# Autodesk Inventor assembly: Pass_Fail_Rig_v2
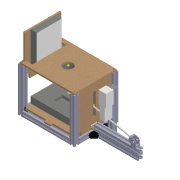
[picture p0: Inventor's stored thumbnail of the model, 180x180]
Saved by Autodesk Inventor 2021 (Build 250183000, 183)
## iProperties
Created: 2021-02-17
Part Number: Pass_Fail_Rig_v2
Document SubType Name: Assembly
Designer: negt20
Author: negt20
## Documents named in this file (23)
- C:\Users\negt20\OneDrive - University of Bath\Documents\Inventor\Pass_Fail_Rig\New Rig\Pass_Fail_Rig_v2.iam
- C:\Users\negt20\OneDrive - University of Bath\Documents\Inventor\Pass_Fail_Rig\New Rig\Strut_Profile_20x20_width.ipt
- C:\Users\negt20\OneDrive - University of Bath\Documents\Inventor\Pass_Fail_Rig\New Rig\Strut_Profile_20x20_height.ipt
- C:\Users\negt20\OneDrive - University of Bath\Documents\Inventor\Pass_Fail_Rig\New Rig\Strut_Profile_20x20_length.ipt
- C:\Users\negt20\OneDrive - University of Bath\Documents\Inventor\Pass_Fail_Rig\New Rig\Inner_Bracket_6mm.ipt
- C:\Users\negt20\OneDrive - University of Bath\Documents\Inventor\Pass_Fail_Rig\New Rig\Outer_Bracket_20x20.ipt
- C:\Users\negt20\OneDrive - University of Bath\Documents\Inventor\Pass_Fail_Rig\New Rig\Strut_Profile_20x20_pivotlength.ipt
- C:\Users\negt20\OneDrive - University of Bath\Documents\Inventor\Pass_Fail_Rig\New Rig\MDF_Hammer_Side.ipt
- C:\Users\negt20\OneDrive - University of Bath\Documents\Inventor\Pass_Fail_Rig\New Rig\Threaded hammer.ipt
- C:\Users\negt20\OneDrive - University of Bath\Documents\Inventor\Pass_Fail_Rig\New Rig\MDF_Side.ipt
- C:\Users\negt20\OneDrive - University of Bath\Documents\Inventor\Pass_Fail_Rig\New Rig\MDF_Front.ipt
- C:\Users\negt20\OneDrive - University of Bath\Documents\Inventor\Pass_Fail_Rig\New Rig\MDF_Base.ipt
- C:\Users\negt20\OneDrive - University of Bath\Documents\Inventor\Pass_Fail_Rig\New Rig\Foam_Side.ipt
- C:\Users\negt20\OneDrive - University of Bath\Documents\Inventor\Pass_Fail_Rig\New Rig\Foam_Hammer_Side.ipt
- C:\Users\negt20\OneDrive - University of Bath\Documents\Inventor\Pass_Fail_Rig\New Rig\Foam_Front.ipt
- C:\Users\negt20\OneDrive - University of Bath\Documents\Inventor\Pass_Fail_Rig\New Rig\Foam_Base.ipt
- C:\Users\negt20\OneDrive - University of Bath\Documents\Inventor\Pass_Fail_Rig\New Rig\MDF_Top_Big_Mic.ipt
- C:\Users\negt20\OneDrive - University of Bath\Documents\Inventor\Pass_Fail_Rig\New Rig\Foam_Top_Big_Mic.ipt
- C:\Users\negt20\OneDrive - University of Bath\Documents\Inventor\Pass_Fail_Rig\New Rig\MDF_Top_Small_Mics.ipt
- C:\Users\negt20\OneDrive - University of Bath\Documents\Inventor\Pass_Fail_Rig\New Rig\Foam_Top_Small_Mics.ipt
- C:\Users\negt20\OneDrive - University of Bath\Documents\Inventor\Pass_Fail_Rig\New Rig\T_NUT_N6.ipt
- C:\Users\negt20\OneDrive - University of Bath\Documents\Inventor\Pass_Fail_Rig\New Rig\Actuator.ipt
- C:\Users\negt20\OneDrive - University of Bath\Documents\Inventor\Pass_Fail_Rig\New Rig\JOINT_20X20_detail.iam
## Components (57 placed, 22 different names)
1. Outer_Bracket_20x20:9 — Mate:104, Mate:105
2. Outer_Bracket_20x20:10 — Mate:106, Mate:107
3. Outer_Bracket_20x20:11 — Mate:108, Mate:109
4. Outer_Bracket_20x20:12 — Mate:110, Mate:111
5. Strut_Profile_20x20_height:1 — Mate:1, Flush:1, Flush:2, Flush:7, Mate:13, Mate:15, Mate:36, Flush:17, Mate:49, Mate:52, Mate:53, Mate:55, Mate:57, Mate:71, Insert:4, Insert:8, Mate:88
6. Strut_Profile_20x20_width:1 — Mate:1, Flush:1, Flush:2, Mate:2, Flush:3, Flush:4, Mate:3, Flush:6, Flush:8, Mate:21, Mate:22, Mate:30, Mate:31, Mate:45, Mate:46, Mate:54, Mate:4, Mate:98, Flush:24, Mate:104, Mate:110
7. Strut_Profile_20x20_height:2 — Mate:2, Flush:3, Flush:4, Flush:5, Mate:18, Mate:26, Mate:35, Flush:15, Flush:16, Mate:47, Mate:51, Mate:59, Mate:62, Mate:67, Mate:68, Mate:74, Mate:79, Insert:2, Insert:7, Mate:97
8. Strut_Profile_20x20_length:1 — Mate:3, Flush:5, Flush:6, Mate:6, Flush:11, Flush:12, Mate:23, Mate:24, Mate:32, Mate:34, Mate:61
9. Strut_Profile_20x20_length:2 — Mate:4, Flush:7, Flush:8, Mate:5, Flush:9, Flush:10, Mate:19, Mate:20, Mate:27, Mate:29, Flush:18, Mate:58, Mate:66
10. Strut_Profile_20x20_height:3 — Mate:5, Flush:9, Flush:10, Mate:7, Mate:11, Mate:12, Mate:56, Mate:63, Mate:64, Insert:3, Insert:5, Mate:96
11. Strut_Profile_20x20_height:4 — Mate:6, Flush:11, Flush:12, Mate:8, Flush:13, Flush:14, Mate:16, Mate:17, Mate:60, Mate:78, Insert:1, Insert:6, Mate:95
12. Strut_Profile_20x20_width:2 — Mate:7, Mate:8, Flush:13, Flush:14, Mate:10, Mate:25, Mate:28, Mate:33, Mate:65-door
13. T_NUT_N6:1 — Insert:9
14. T_NUT_N6:2 — Insert:12
15. T_NUT_N6:3 — Insert:10
16. T_NUT_N6:4 — Insert:11
17. Inner_Bracket_6mm:1 — Mate:10, Mate:11, Mate:96
18. Inner_Bracket_6mm:2 — Mate:13, Mate:22
19. Inner_Bracket_6mm:3 — Mate:12, Mate:20
20. Inner_Bracket_6mm:4 — Mate:16, Mate:24, Mate:78
21. Inner_Bracket_6mm:5 — Mate:17, Mate:25, Mate:95
22. Inner_Bracket_6mm:6 — Mate:18, Mate:21
23. Inner_Bracket_6mm:7 — Mate:15, Mate:19
24. Inner_Bracket_6mm:8 — Mate:23, Mate:26, Mate:79
25. Outer_Bracket_20x20:1 — Mate:27, Mate:28
26. Outer_Bracket_20x20:2 — Mate:29, Mate:30
27. Outer_Bracket_20x20:3 — Mate:31, Mate:32
28. Outer_Bracket_20x20:4 — Mate:33, Mate:34
29. MDF_Top_Big_Mic:1 — Insert:1, Insert:2, Insert:3, Insert:4, Mate:86
30. MDF_Top_Small_Mics:1 — Insert:5, Insert:6, Insert:7, Insert:8, Mate:88
31. MDF_Base:1 — Mate:66, Mate:67, Mate:68, Mate:70, Mate:73, Mate:76, Mate:83, Insert:9, Insert:10, Insert:11, Insert:12
32. MDF_Side:1 — Mate:55, Mate:56, Mate:57, Mate:58, Mate:69
33. MDF_Hammer_Side:1 — Mate:51, Mate:52, Mate:53, Mate:54, Mate:75, Flush:27
34. MDF_Front:1 — Mate:63, Mate:64, Mate:65-door, Mate:80, Flush:22
35. MDF_Side:2 — Mate:59, Mate:60, Mate:61, Mate:62, Mate:72
36. Foam_Top_Big_Mic:1 — Mate:86, Mate:87, Mate:91
37. Foam_Top_Small_Mics:1 — Mate:89, Mate:90, Flush:23
38. Foam_Base:1 — Mate:83, Mate:84, Mate:93
39. Foam_Side:1 — Mate:69, Mate:70, Mate:71, Mate:90, Mate:91, Mate:92, Mate:93, Mate:94
40. Foam_Hammer_Side:1 — Mate:75, Mate:76, Mate:84, Mate:87, Mate:89, Flush:23, Mate:94
41. Foam_Front:1 — Mate:80, Flush:22, Mate:92
42. Foam_Side:2 — Mate:72, Mate:73, Mate:74
43. Strut_Profile_20x20_pivotlength:1 — Mate:35, Flush:15, Flush:16, Mate:37, Flush:19, Flush:20, Mate:39, Mate:41, Mate:48
44. Strut_Profile_20x20_pivotlength:2 — Mate:36, Flush:17, Flush:18, Mate:38, Mate:40, Mate:42, Mate:50
45. Strut_Profile_20x20_width:3 — Mate:37, Mate:38, Flush:19, Flush:20, Mate:43, Mate:44
46. Outer_Bracket_20x20:5 — Mate:40, Mate:45
47. Outer_Bracket_20x20:6 — Mate:39, Mate:46
48. Outer_Bracket_20x20:7 — Mate:41, Mate:43
49. Outer_Bracket_20x20:8 — Mate:42, Mate:44
50. Inner_Bracket_6mm:9 — Mate:49, Mate:50
51. Inner_Bracket_6mm:10 — Mate:47, Mate:48, Mate:97
52. Threaded hammer:1 — Insert:13, Mate:103
53. Strut_Profile_20x20_pivotlength:3 — Mate:98, Flush:24, Mate:99, Flush:25, Flush:27, Flush:28, Flush:29, Mate:101, Mate:105, Mate:107, Mate:111
54. Strut_Profile_20x20_height:5 — Mate:99, Flush:25, Mate:100, Flush:26, Mate:106, Mate:109
55. Actuator:1 — Mate:100, Flush:26
56. Strut_Profile_20x20_pivotlength:4 — Flush:28, Flush:29, Mate:101, Mate:102, Mate:108
57. JOINT_20X20_detail:1 [sub-assembly] — Mate:102, Insert:13, Mate:103
## Relationships (146: Mate 105, Flush 28, Insert 13)
- Mate:1: Strut_Profile_20x20_height:1 ↔ Strut_Profile_20x20_width:1
- Flush:1: Strut_Profile_20x20_height:1 ↔ Strut_Profile_20x20_width:1
- Flush:2: Strut_Profile_20x20_height:1 ↔ Strut_Profile_20x20_width:1
- Mate:2: Strut_Profile_20x20_width:1 ↔ Strut_Profile_20x20_height:2
- Flush:3: Strut_Profile_20x20_width:1 ↔ Strut_Profile_20x20_height:2
- Flush:4: Strut_Profile_20x20_width:1 ↔ Strut_Profile_20x20_height:2
- Mate:3: Strut_Profile_20x20_width:1 ↔ Strut_Profile_20x20_length:1
- Flush:5: Strut_Profile_20x20_height:2 ↔ Strut_Profile_20x20_length:1
- Flush:6: Strut_Profile_20x20_width:1 ↔ Strut_Profile_20x20_length:1
- Mate:4: Strut_Profile_20x20_width:1 ↔ Strut_Profile_20x20_length:2
- Flush:7: Strut_Profile_20x20_height:1 ↔ Strut_Profile_20x20_length:2
- Flush:8: Strut_Profile_20x20_width:1 ↔ Strut_Profile_20x20_length:2
- Mate:5: Strut_Profile_20x20_length:2 ↔ Strut_Profile_20x20_height:3
- Flush:9: Strut_Profile_20x20_length:2 ↔ Strut_Profile_20x20_height:3
- Flush:10: Strut_Profile_20x20_length:2 ↔ Strut_Profile_20x20_height:3
- Mate:6: Strut_Profile_20x20_length:1 ↔ Strut_Profile_20x20_height:4
- Flush:11: Strut_Profile_20x20_length:1 ↔ Strut_Profile_20x20_height:4
- Flush:12: Strut_Profile_20x20_length:1 ↔ Strut_Profile_20x20_height:4
- Mate:7: Strut_Profile_20x20_height:3 ↔ Strut_Profile_20x20_width:2
- Mate:8: Strut_Profile_20x20_height:4 ↔ Strut_Profile_20x20_width:2
- Flush:13: Strut_Profile_20x20_height:4 ↔ Strut_Profile_20x20_width:2
- Flush:14: Strut_Profile_20x20_height:4 ↔ Strut_Profile_20x20_width:2
- Mate:10: Strut_Profile_20x20_width:2 ↔ Inner_Bracket_6mm:1
- Mate:11: Strut_Profile_20x20_height:3 ↔ Inner_Bracket_6mm:1
- Mate:12: Strut_Profile_20x20_height:3 ↔ Inner_Bracket_6mm:3
- Mate:13: Strut_Profile_20x20_height:1 ↔ Inner_Bracket_6mm:2
- Mate:15: Strut_Profile_20x20_height:1 ↔ Inner_Bracket_6mm:7
- Mate:16: Strut_Profile_20x20_height:4 ↔ Inner_Bracket_6mm:4
- Mate:17: Strut_Profile_20x20_height:4 ↔ Inner_Bracket_6mm:5
- Mate:18: Strut_Profile_20x20_height:2 ↔ Inner_Bracket_6mm:6
- Mate:19: Strut_Profile_20x20_length:2 ↔ Inner_Bracket_6mm:7
- Mate:20: Strut_Profile_20x20_length:2 ↔ Inner_Bracket_6mm:3
- Mate:21: Strut_Profile_20x20_width:1 ↔ Inner_Bracket_6mm:6
- Mate:22: Strut_Profile_20x20_width:1 ↔ Inner_Bracket_6mm:2
- Mate:23: Strut_Profile_20x20_length:1 ↔ Inner_Bracket_6mm:8
- Mate:24: Strut_Profile_20x20_length:1 ↔ Inner_Bracket_6mm:4
- Mate:25: Strut_Profile_20x20_width:2 ↔ Inner_Bracket_6mm:5
- Mate:26: Strut_Profile_20x20_height:2 ↔ Inner_Bracket_6mm:8
- Mate:27: Strut_Profile_20x20_length:2 ↔ Outer_Bracket_20x20:1
- Mate:28: Strut_Profile_20x20_width:2 ↔ Outer_Bracket_20x20:1
- Mate:29: Strut_Profile_20x20_length:2 ↔ Outer_Bracket_20x20:2
- Mate:30: Strut_Profile_20x20_width:1 ↔ Outer_Bracket_20x20:2
- Mate:31: Strut_Profile_20x20_width:1 ↔ Outer_Bracket_20x20:3
- Mate:32: Strut_Profile_20x20_length:1 ↔ Outer_Bracket_20x20:3
- Mate:33: Strut_Profile_20x20_width:2 ↔ Outer_Bracket_20x20:4
- Mate:34: Strut_Profile_20x20_length:1 ↔ Outer_Bracket_20x20:4
- Mate:35: Strut_Profile_20x20_height:2 ↔ Strut_Profile_20x20_pivotlength:1
- Flush:15: Strut_Profile_20x20_height:2 ↔ Strut_Profile_20x20_pivotlength:1
- Flush:16: Strut_Profile_20x20_height:2 ↔ Strut_Profile_20x20_pivotlength:1
- Mate:36: Strut_Profile_20x20_height:1 ↔ Strut_Profile_20x20_pivotlength:2
- Flush:17: Strut_Profile_20x20_height:1 ↔ Strut_Profile_20x20_pivotlength:2
- Flush:18: Strut_Profile_20x20_length:2 ↔ Strut_Profile_20x20_pivotlength:2
- Mate:37: Strut_Profile_20x20_pivotlength:1 ↔ Strut_Profile_20x20_width:3
- Mate:38: Strut_Profile_20x20_pivotlength:2 ↔ Strut_Profile_20x20_width:3
- Flush:19: Strut_Profile_20x20_pivotlength:1 ↔ Strut_Profile_20x20_width:3
- Flush:20: Strut_Profile_20x20_pivotlength:1 ↔ Strut_Profile_20x20_width:3
- Mate:39: Strut_Profile_20x20_pivotlength:1 ↔ Outer_Bracket_20x20:6
- Mate:40: Strut_Profile_20x20_pivotlength:2 ↔ Outer_Bracket_20x20:5
- Mate:41: Strut_Profile_20x20_pivotlength:1 ↔ Outer_Bracket_20x20:7
- Mate:42: Strut_Profile_20x20_pivotlength:2 ↔ Outer_Bracket_20x20:8
- Mate:43: Strut_Profile_20x20_width:3 ↔ Outer_Bracket_20x20:7
- Mate:44: Strut_Profile_20x20_width:3 ↔ Outer_Bracket_20x20:8
- Mate:45: Strut_Profile_20x20_width:1 ↔ Outer_Bracket_20x20:5
- Mate:46: Strut_Profile_20x20_width:1 ↔ Outer_Bracket_20x20:6
- Mate:47: Strut_Profile_20x20_height:2 ↔ Inner_Bracket_6mm:10
- Mate:48: Strut_Profile_20x20_pivotlength:1 ↔ Inner_Bracket_6mm:10
- Mate:49: Strut_Profile_20x20_height:1 ↔ Inner_Bracket_6mm:9
- Mate:50: Strut_Profile_20x20_pivotlength:2 ↔ Inner_Bracket_6mm:9
- Mate:51: Strut_Profile_20x20_height:2 ↔ MDF_Hammer_Side:1
- Mate:52: Strut_Profile_20x20_height:1 ↔ MDF_Hammer_Side:1
- Mate:53: Strut_Profile_20x20_height:1 ↔ MDF_Hammer_Side:1
- Mate:54: Strut_Profile_20x20_width:1 ↔ MDF_Hammer_Side:1
- Mate:55: Strut_Profile_20x20_height:1 ↔ MDF_Side:1
- Mate:56: Strut_Profile_20x20_height:3 ↔ MDF_Side:1
- Mate:57: Strut_Profile_20x20_height:1 ↔ MDF_Side:1
- Mate:58: Strut_Profile_20x20_length:2 ↔ MDF_Side:1
- Mate:59: Strut_Profile_20x20_height:2 ↔ MDF_Side:2
- Mate:60: Strut_Profile_20x20_height:4 ↔ MDF_Side:2
- Mate:61: Strut_Profile_20x20_length:1 ↔ MDF_Side:2
- Mate:62: Strut_Profile_20x20_height:2 ↔ MDF_Side:2
- Mate:63: Strut_Profile_20x20_height:3 ↔ MDF_Front:1
- Mate:64 (0.5 mm): Strut_Profile_20x20_height:3 ↔ MDF_Front:1
- Mate:65-door (100 mm): Strut_Profile_20x20_width:2 ↔ MDF_Front:1
- Mate:66: Strut_Profile_20x20_length:2 ↔ MDF_Base:1
- Mate:67: Strut_Profile_20x20_height:2 ↔ MDF_Base:1
- Mate:68: Strut_Profile_20x20_height:2 ↔ MDF_Base:1
- Mate:69: MDF_Side:1 ↔ Foam_Side:1
- Mate:70: MDF_Base:1 ↔ Foam_Side:1
- Mate:71: Strut_Profile_20x20_height:1 ↔ Foam_Side:1
- Mate:72: MDF_Side:2 ↔ Foam_Side:2
- Mate:73: MDF_Base:1 ↔ Foam_Side:2
- Mate:74: Strut_Profile_20x20_height:2 ↔ Foam_Side:2
- Mate:75: MDF_Hammer_Side:1 ↔ Foam_Hammer_Side:1
- Mate:76: MDF_Base:1 ↔ Foam_Hammer_Side:1
- Mate:78: Strut_Profile_20x20_height:4 ↔ Inner_Bracket_6mm:4
- Mate:79: Strut_Profile_20x20_height:2 ↔ Inner_Bracket_6mm:8
- Mate:80: MDF_Front:1 ↔ Foam_Front:1
- Mate:83: MDF_Base:1 ↔ Foam_Base:1
- Mate:84: Foam_Base:1 ↔ Foam_Hammer_Side:1
- Insert:1: Strut_Profile_20x20_height:4 ↔ MDF_Top_Big_Mic:1
- Insert:2: Strut_Profile_20x20_height:2 ↔ MDF_Top_Big_Mic:1
- Insert:3: Strut_Profile_20x20_height:3 ↔ MDF_Top_Big_Mic:1
- Insert:4: Strut_Profile_20x20_height:1 ↔ MDF_Top_Big_Mic:1
- Mate:86: MDF_Top_Big_Mic:1 ↔ Foam_Top_Big_Mic:1
- Mate:87: Foam_Top_Big_Mic:1 ↔ Foam_Hammer_Side:1
- Flush:22: MDF_Front:1 ↔ Foam_Front:1
- Insert:5: Strut_Profile_20x20_height:3 ↔ MDF_Top_Small_Mics:1
- Insert:6: Strut_Profile_20x20_height:4 ↔ MDF_Top_Small_Mics:1
- Insert:7: Strut_Profile_20x20_height:2 ↔ MDF_Top_Small_Mics:1
- Insert:8: Strut_Profile_20x20_height:1 ↔ MDF_Top_Small_Mics:1
- Mate:88: Strut_Profile_20x20_height:1 ↔ MDF_Top_Small_Mics:1
- Mate:89: Foam_Top_Small_Mics:1 ↔ Foam_Hammer_Side:1
- Mate:90: Foam_Top_Small_Mics:1 ↔ Foam_Side:1
- Flush:23: Foam_Top_Small_Mics:1 ↔ Foam_Hammer_Side:1
- Mate:91: Foam_Top_Big_Mic:1 ↔ Foam_Side:1
- Mate:92: Foam_Side:1 ↔ Foam_Front:1
- Mate:93: Foam_Base:1 ↔ Foam_Side:1
- Mate:94: Foam_Side:1 ↔ Foam_Hammer_Side:1
- Mate:95: Strut_Profile_20x20_height:4 ↔ Inner_Bracket_6mm:5
- Mate:96: Strut_Profile_20x20_height:3 ↔ Inner_Bracket_6mm:1
- Insert:9: T_NUT_N6:1 ↔ MDF_Base:1
- Insert:10: T_NUT_N6:3 ↔ MDF_Base:1
- Insert:11: T_NUT_N6:4 ↔ MDF_Base:1
- Insert:12: T_NUT_N6:2 ↔ MDF_Base:1
- Mate:97: Strut_Profile_20x20_height:2 ↔ Inner_Bracket_6mm:10
- Mate:98: Strut_Profile_20x20_width:1 ↔ Strut_Profile_20x20_pivotlength:3
- Flush:24: Strut_Profile_20x20_width:1 ↔ Strut_Profile_20x20_pivotlength:3
- Mate:99: Strut_Profile_20x20_pivotlength:3 ↔ Strut_Profile_20x20_height:5
- Flush:25: Strut_Profile_20x20_pivotlength:3 ↔ Strut_Profile_20x20_height:5
- Mate:100: Strut_Profile_20x20_height:5 ↔ Actuator:1
- Flush:26: Strut_Profile_20x20_height:5 ↔ Actuator:1
- Flush:27 (-2 mm): MDF_Hammer_Side:1 ↔ Strut_Profile_20x20_pivotlength:3
- Flush:28: Strut_Profile_20x20_pivotlength:3 ↔ Strut_Profile_20x20_pivotlength:4
- Flush:29: Strut_Profile_20x20_pivotlength:3 ↔ Strut_Profile_20x20_pivotlength:4
- Mate:101: Strut_Profile_20x20_pivotlength:3 ↔ Strut_Profile_20x20_pivotlength:4
- Mate:102: Strut_Profile_20x20_pivotlength:4 ↔ JOINT_20X20_detail:1
- Insert:13: Threaded hammer:1 ↔ JOINT_20X20_detail:1
- Mate:103: Threaded hammer:1 ↔ JOINT_20X20_detail:1
- Mate:104: Outer_Bracket_20x20:9 ↔ Strut_Profile_20x20_width:1
- Mate:105: Outer_Bracket_20x20:9 ↔ Strut_Profile_20x20_pivotlength:3
- Mate:106: Outer_Bracket_20x20:10 ↔ Strut_Profile_20x20_height:5
- Mate:107: Outer_Bracket_20x20:10 ↔ Strut_Profile_20x20_pivotlength:3
- Mate:108: Outer_Bracket_20x20:11 ↔ Strut_Profile_20x20_pivotlength:4
- Mate:109: Outer_Bracket_20x20:11 ↔ Strut_Profile_20x20_height:5
- Mate:110: Outer_Bracket_20x20:12 ↔ Strut_Profile_20x20_width:1
- Mate:111: Outer_Bracket_20x20:12 ↔ Strut_Profile_20x20_pivotlength:3
